# Autodesk Inventor assembly: MSAL 32 50
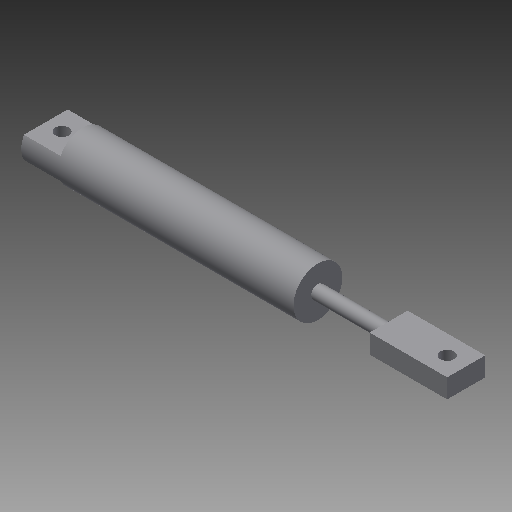
[picture p0: Inventor's stored thumbnail of the model, 512x512]
Saved by Autodesk Inventor 2019.4 (Build 234330000, 330)
## iProperties
Created: 2020-01-02
Part Number: MSAL 32 50
Document SubType Name: Assembly
Designer: Mark
Author: Mark
## Documents named in this file (3)
- C:\Users\Mark\Desktop\7738 Helion Engineering\7738-CAD-prep\Butterfly Drive Mk3\MSAL 32 50.iam
- C:\Users\Mark\Desktop\7738 Helion Engineering\7738-CAD-prep\Butterfly Drive Mk3\MSAL 32 50 Stand In.ipt
- C:\Users\Mark\Desktop\7738 Helion Engineering\7738-CAD-prep\Butterfly Drive Mk3\MSAL Pushing Thing.ipt
## Components (2 placed, 2 different names)
1. MTAL 32 50 Stand In:1 — Cylindrical:1
2. MTAL Pushing Thing:1 — Cylindrical:1
## Relationships (1: CylindricalJoint 1)
- Cylindrical:1: MTAL 32 50 Stand In:1 ↔ MTAL Pushing Thing:1
